# Autodesk Inventor assembly: FingerGeneric
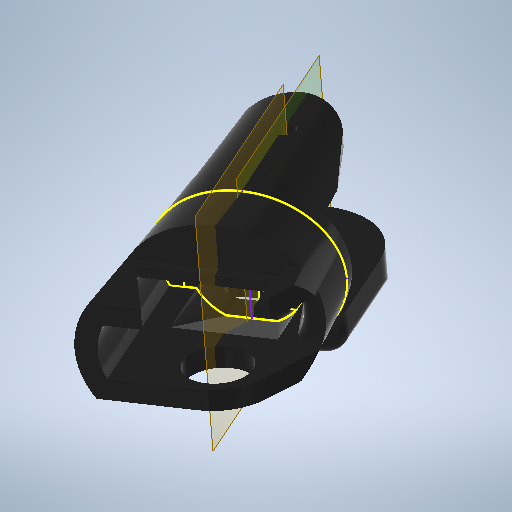
[picture p0: Inventor's stored thumbnail of the model, 512x512]
Saved by Autodesk Inventor 2025.1 (Build 291241000, 241)
## iProperties
Created: 2024-09-11
Part Number: FingerGeneric
Document SubType Name: Assembly
Designer: Alexander
Author: Alexander
## Documents named in this file (3)
- D:\Repositorios_Politecnica\Handi-EPN\CAD\Sim Models\GenericMiddlePhalanx.iam
- D:\Repositorios_Politecnica\Handi-EPN\CAD\Right Finger\IP - D R.ipt
- D:\Repositorios_Politecnica\Handi-EPN\CAD\Right Finger\IP - P Main R.ipt
## Components (2 placed, 2 different names)
1. IP - D R:1 — Mate:1, Mate:2, Flush:4
2. IP - P Main R:1 — Flush:1, Flush:2, Flush:3, Mate:1, Mate:2, Flush:4
## Relationships (6: Flush 4, Mate 2)
- Flush:1: IP - P Main R:1
- Flush:2: IP - P Main R:1
- Flush:3: IP - P Main R:1
- Mate:1: IP - D R:1 ↔ IP - P Main R:1
- Mate:2: IP - D R:1 ↔ IP - P Main R:1
- Flush:4 (2.2 mm): IP - D R:1 ↔ IP - P Main R:1
